# Autodesk Inventor assembly: ExampleServoAssembly
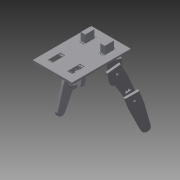
[picture p0: Inventor's stored thumbnail of the model, 180x180]
Saved by Autodesk Inventor 2014 SP1 (Build 180222100, 222)
## iProperties
Created: 2014-01-19
Part Number: ExampleServoAssembly
Document SubType Name: Assembly
Designer: david
Author: david
## Documents named in this file (12)
- C:\Users\asus\Documents\Autodesk\Projects\SheepWarrior\SheepBot.iam
- C:\Users\asus\Documents\Autodesk\Projects\RobotsWar\Docs\3D\CommonComponents\SimplifiedServo.ipt
- C:\Users\asus\Documents\Autodesk\Projects\RobotsWar\Docs\3D\CommonComponents\SimplifiedServoArm.ipt
- C:\Users\asus\Documents\Autodesk\Projects\SheepWarrior\LegParts\FrontLowerLeg.ipt
- C:\Users\asus\Documents\Autodesk\Projects\SheepWarrior\LegParts\FrontUpperLeg.ipt
- C:\Users\asus\Documents\Autodesk\Projects\SheepWarrior\LegParts\FrontUpperLegShoulder.ipt
- C:\Users\asus\Documents\Autodesk\Projects\RobotsWar\Docs\3D\CommonComponents\SimplifiedServo_MIR.ipt
- C:\Users\asus\Documents\Autodesk\Projects\RobotsWar\Docs\3D\CommonComponents\SimplifiedServoArm_MIR.ipt
- C:\Users\asus\Documents\Autodesk\Projects\SheepWarrior\LegParts\FrontLowerLeg_MIR.ipt
- C:\Users\asus\Documents\Autodesk\Projects\SheepWarrior\LegParts\FrontUpperLeg_MIR.ipt
- C:\Users\asus\Documents\Autodesk\Projects\SheepWarrior\LegParts\FrontUpperLegShoulder_MIR.ipt
- C:\Users\asus\Documents\Autodesk\Projects\SheepWarrior\SheepBody.ipt
## Components (19 placed, 11 different names)
1. SimplifiedServo:1 — Rotational:1, Insert:1, Mate:7, Mate:8, Mate:9
2. SimplifiedServoArm:1 — Rotational:1, Mate:1, Angle:1
3. FrontLowerLeg:1 — Mate:1, Insert:1, Angle:1
4. FrontUpperLeg:1 — Mate:5, Mate:6, Angle:2, Mate:7, Mate:8, Mate:9
5. SimplifiedServoArm:2 — Mate:5, Mate:6, Angle:2, Rotational:2
6. SimplifiedServo:2 — Rotational:2, Mate:10, Mate:11, Mate:12
7. FrontUpperLegShoulder:1 — Mate:10, Mate:11, Mate:12, Mate:13, Mate:14, Angle:3
8. SimplifiedServoArm:3 — Rotational:3, Mate:13, Mate:14, Angle:3
9. SimplifiedServo:3 — Rotational:3, Mate:26, Mate:27, Mate:28
10. SimplifiedServo_MIR:1 — Insert:2, Mate:16, Mate:17, Mate:18, Rotational:4
11. SimplifiedServoArm_MIR:1 — Mate:15, Angle:4, Rotational:4
12. FrontLowerLeg_MIR:1 — Insert:2, Mate:15, Angle:4
13. FrontUpperLeg_MIR:1 — Mate:16, Mate:17, Mate:18, Mate:19, Mate:20, Angle:5
14. SimplifiedServoArm_MIR:2 — Mate:19, Mate:20, Angle:5, Rotational:5
15. SimplifiedServo_MIR:2 — Mate:21, Mate:22, Mate:23, Rotational:5
16. FrontUpperLegShoulder_MIR:1 — Mate:21, Mate:22, Mate:23, Mate:24, Mate:25, Angle:6
17. SimplifiedServoArm_MIR:3 — Mate:24, Mate:25, Angle:6, Rotational:6
18. SimplifiedServo_MIR:3 — Rotational:6, Mate:29, Mate:30, Mate:31
19. SheepBody:1 — Mate:26, Mate:27, Mate:28, Mate:29, Mate:30, Mate:31
## Relationships (42: Mate 28, RevoluteJoint 6, Angle 6, Insert 2)
- Rotational:1 [RevoluteJoint]: SimplifiedServo:1 ↔ SimplifiedServoArm:1
- Mate:1: SimplifiedServoArm:1 ↔ FrontLowerLeg:1
- Insert:1: SimplifiedServo:1 ↔ FrontLowerLeg:1
- Angle:1 (0 deg): SimplifiedServoArm:1 ↔ FrontLowerLeg:1
- Mate:5: FrontUpperLeg:1 ↔ SimplifiedServoArm:2
- Mate:6: FrontUpperLeg:1 ↔ SimplifiedServoArm:2
- Angle:2 (0 deg): FrontUpperLeg:1 ↔ SimplifiedServoArm:2
- Rotational:2 [RevoluteJoint]: SimplifiedServoArm:2 ↔ SimplifiedServo:2
- Mate:7: SimplifiedServo:1 ↔ FrontUpperLeg:1
- Mate:8: SimplifiedServo:1 ↔ FrontUpperLeg:1
- Mate:9: SimplifiedServo:1 ↔ FrontUpperLeg:1
- Mate:10: SimplifiedServo:2 ↔ FrontUpperLegShoulder:1
- Mate:11: SimplifiedServo:2 ↔ FrontUpperLegShoulder:1
- Mate:12: SimplifiedServo:2 ↔ FrontUpperLegShoulder:1
- Rotational:3 [RevoluteJoint]: SimplifiedServoArm:3 ↔ SimplifiedServo:3
- Mate:13: FrontUpperLegShoulder:1 ↔ SimplifiedServoArm:3
- Mate:14: FrontUpperLegShoulder:1 ↔ SimplifiedServoArm:3
- Angle:3 (0 deg): FrontUpperLegShoulder:1 ↔ SimplifiedServoArm:3
- Insert:2: SimplifiedServo_MIR:1 ↔ FrontLowerLeg_MIR:1
- Mate:15: SimplifiedServoArm_MIR:1 ↔ FrontLowerLeg_MIR:1
- Angle:4 (0 deg): SimplifiedServoArm_MIR:1 ↔ FrontLowerLeg_MIR:1
- Mate:16: SimplifiedServo_MIR:1 ↔ FrontUpperLeg_MIR:1
- Mate:17: SimplifiedServo_MIR:1 ↔ FrontUpperLeg_MIR:1
- Mate:18: SimplifiedServo_MIR:1 ↔ FrontUpperLeg_MIR:1
- Mate:19: FrontUpperLeg_MIR:1 ↔ SimplifiedServoArm_MIR:2
- Mate:20: FrontUpperLeg_MIR:1 ↔ SimplifiedServoArm_MIR:2
- Angle:5 (0 deg): FrontUpperLeg_MIR:1 ↔ SimplifiedServoArm_MIR:2
- Mate:21: SimplifiedServo_MIR:2 ↔ FrontUpperLegShoulder_MIR:1
- Mate:22: SimplifiedServo_MIR:2 ↔ FrontUpperLegShoulder_MIR:1
- Mate:23: SimplifiedServo_MIR:2 ↔ FrontUpperLegShoulder_MIR:1
- Mate:24: FrontUpperLegShoulder_MIR:1 ↔ SimplifiedServoArm_MIR:3
- Mate:25: FrontUpperLegShoulder_MIR:1 ↔ SimplifiedServoArm_MIR:3
- Angle:6 (0 deg): FrontUpperLegShoulder_MIR:1 ↔ SimplifiedServoArm_MIR:3
- Rotational:4 [RevoluteJoint]: SimplifiedServo_MIR:1 ↔ SimplifiedServoArm_MIR:1
- Rotational:5 [RevoluteJoint]: SimplifiedServoArm_MIR:2 ↔ SimplifiedServo_MIR:2
- Rotational:6 [RevoluteJoint]: SimplifiedServoArm_MIR:3 ↔ SimplifiedServo_MIR:3
- Mate:26: SimplifiedServo:3 ↔ SheepBody:1
- Mate:27: SimplifiedServo:3 ↔ SheepBody:1
- Mate:28: SimplifiedServo:3 ↔ SheepBody:1
- Mate:29: SimplifiedServo_MIR:3 ↔ SheepBody:1
- Mate:30: SimplifiedServo_MIR:3 ↔ SheepBody:1
- Mate:31: SimplifiedServo_MIR:3 ↔ SheepBody:1
